# Autodesk Inventor assembly: Montagem3
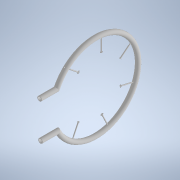
[picture p0: Inventor's stored thumbnail of the model, 180x180]
Saved by Autodesk Inventor 2021 (Build 250183000, 183)
## iProperties
Created: 2021-07-26
Part Number: Montagem3
Document SubType Name: Assembly
Designer: Giovanni
Author: Giovanni
## Documents named in this file (4)
- C:\Users\irineu\Documents\Inventor\MotorRadial7\Montagem3.iam
- C:\Users\irineu\Documents\Inventor\MotorRadial7\Peça46.ipt
- C:\Users\irineu\Documents\Inventor\MotorRadial7\Peça47.ipt
- C:\Users\irineu\Documents\Inventor\MotorRadial7\Tubo auxiliar 1.iam
## Components (13 placed, 3 different names)
1. Peça46:1 — Coincidente:1, Coincidente:2, Coincidente:3, Coincidente:4, Coincidente:5, Coincidente:6
2. Peça47:1 — Coincidente:1, Inserir:2
3. Peça47:2 — Coincidente:2, Inserir:1
4. Peça47:3 — Coincidente:3, Inserir:3
5. Peça47:4 — Coincidente:4, Inserir:4
6. Peça47:5 — Coincidente:5, Inserir:5
7. Peça47:6 — Coincidente:6, Inserir:6
8. Tubo auxiliar 1:1 [sub-assembly] — Inserir:1
9. Tubo auxiliar 1:2 [sub-assembly] — Inserir:2
10. Tubo auxiliar 1:3 [sub-assembly] — Inserir:3
11. Tubo auxiliar 1:4 [sub-assembly] — Inserir:4
12. Tubo auxiliar 1:5 [sub-assembly] — Inserir:6
13. Tubo auxiliar 1:6 [sub-assembly] — Inserir:5
## Relationships (12: Mate 6, Insert 6)
- Coincidente:1 [Mate]: Peça46:1 ↔ Peça47:1
- Coincidente:2 [Mate]: Peça46:1 ↔ Peça47:2
- Coincidente:3 [Mate]: Peça46:1 ↔ Peça47:3
- Coincidente:4 [Mate]: Peça46:1 ↔ Peça47:4
- Coincidente:5 [Mate]: Peça46:1 ↔ Peça47:5
- Coincidente:6 [Mate]: Peça46:1 ↔ Peça47:6
- Inserir:1: Peça47:2 ↔ Tubo auxiliar 1:1
- Inserir:2: Peça47:1 ↔ Tubo auxiliar 1:2
- Inserir:3: Peça47:3 ↔ Tubo auxiliar 1:3
- Inserir:4: Peça47:4 ↔ Tubo auxiliar 1:4
- Inserir:5: Peça47:5 ↔ Tubo auxiliar 1:6
- Inserir:6: Peça47:6 ↔ Tubo auxiliar 1:5
